# Autodesk Inventor assembly: folivora
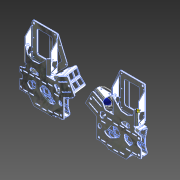
[picture p0: Inventor's stored thumbnail of the model, 180x180]
Saved by Autodesk Inventor 2018 (Build 220112000, 112)
## iProperties
Created: 2018-05-16
Part Number: folivora
Material: 一般
Document SubType Name: Assembly
Designer: NaMACHAN
Mass: 637.628 g
Surface Area: 2506.17 cm^2
Volume: 247.109 cm^3
Density: 2.58035 g/cm^3
Author: NaMACHAN
## Documents named in this file (25)
- C:\Users\NaMACHAN\Dropbox\Project\original\folivora\inventor\folivora.iam
- C:\Users\NaMACHAN\Dropbox\Project\original\folivora\inventor\baseframe.ipt
- C:\Users\NaMACHAN\Dropbox\Project\original\folivora\inventor\keyplate3.ipt
- C:\Users\NaMACHAN\Dropbox\Project\original\folivora\inventor\keyplate4.ipt
- C:\Users\NaMACHAN\Dropbox\Project\original\folivora\inventor\keyL.ipt
- C:\Users\NaMACHAN\Dropbox\Project\original\folivora\inventor\ball.ipt
- C:\Users\NaMACHAN\Dropbox\Project\original\folivora\inventor\trackball-base.ipt
- C:\Users\NaMACHAN\Dropbox\Project\original\folivora\inventor\trackball-shaft.ipt
- C:\Users\NaMACHAN\Dropbox\Project\original\folivora\inventor\bearing.ipt
- C:\Users\NaMACHAN\Dropbox\Project\original\folivora\inventor\bearingcover.ipt
- C:\Users\NaMACHAN\Dropbox\Project\original\folivora\inventor\trackball_l.ipt
- C:\Users\NaMACHAN\Dropbox\Project\original\folivora\inventor\trackball-cover.ipt
- C:\Users\NaMACHAN\Dropbox\Project\original\folivora\inventor\trackball-spacer.ipt
- C:\Users\NaMACHAN\Dropbox\Project\original\folivora\inventor\palmrest.ipt
- C:\Users\NaMACHAN\Dropbox\Project\original\folivora\inventor\palmrest-plate.ipt
- C:\Users\NaMACHAN\Dropbox\Project\original\folivora\inventor\baseframe_left.ipt
- C:\Users\NaMACHAN\Dropbox\Project\original\folivora\inventor\palmrest_left.ipt
- C:\Users\NaMACHAN\Dropbox\Project\original\folivora\inventor\thumbkey_L.ipt
- C:\Users\NaMACHAN\Dropbox\Project\original\folivora\inventor\keyplate2.ipt
- C:\Users\NaMACHAN\Dropbox\Project\original\folivora\inventor\folivora\AIP\FEA\cjjue1qww.fins
- C:\Users\NaMACHAN\Dropbox\Project\original\folivora\inventor\folivora\AIP\FEA\cjjue1qww.fsat
- C:\Users\NaMACHAN\Dropbox\Project\original\folivora\inventor\folivora\AIP\FEA\cjjue1qww.ftes
- C:\Users\NaMACHAN\Dropbox\Project\original\folivora\inventor\folivora\AIP\FEA\cjjue1qww.fwiz
- C:\Users\NaMACHAN\Dropbox\Project\original\folivora\inventor\folivora\AIP\FEA\cjjue1r1c.fmsh
- C:\Users\NaMACHAN\Dropbox\Project\original\folivora\inventor\folivora\AIP\FEA\cjjue1r1d.fres
## Components (61 placed, 18 different names)
1. baseframe:1 — メイト:31, メイト:32, メイト:33, メイト:34, メイト:37, メイト:38, メイト:39, メイト:40, メイト:43, メイト:79, メイト:80, メイト:89, メイト:94, メイト:114, フラッシュ:19, フラッシュ:20, フラッシュ:21, フラッシュ:22, フラッシュ:23, フラッシュ:24, メイト:141, メイト:205, メイト:206, メイト:207
2. keyL:1 — メイト:1, メイト:2, メイト:3, 角度:1, メイト:33
3. keyplate4:1 — メイト:1, メイト:2, メイト:3, メイト:4, メイト:5, 角度:1, メイト:46, メイト:95
4. keyL:2 — メイト:4, メイト:5, メイト:37, メイト:43, フラッシュ:5, フラッシュ:12, フラッシュ:22
5. keyplate3:1 — メイト:6, メイト:7, メイト:8, メイト:9, メイト:10, 角度:2, メイト:44, メイト:45
6. keyL:3 — メイト:7, メイト:10, 角度:2, メイト:32
7. keyL:4 — メイト:6, メイト:8, メイト:9, メイト:40, フラッシュ:3, フラッシュ:4
8. keyplate3:2 — メイト:44
9. keyL:5 — メイト:31
10. keyL:6 — メイト:39, フラッシュ:3
11. keyL:7 — メイト:34
12. keyplate4:2 — メイト:45, メイト:46
13. keyL:8 — メイト:38, フラッシュ:4, フラッシュ:5
14. ball:1 — メイト:105, メイト:115
15. trackball-base:1 — メイト:52, メイト:53, メイト:54, メイト:55, メイト:56, メイト:57, メイト:58, メイト:59, メイト:60, メイト:61, メイト:62, メイト:63, フラッシュ:15, メイト:105, フラッシュ:16, メイト:117, メイト:118, メイト:119, メイト:120, メイト:124, メイト:125
16. trackball-shaft:1 — メイト:49, メイト:52, メイト:53, メイト:54
17. bearing:1 — メイト:49, メイト:55
18. trackball-shaft:2 — メイト:56, メイト:57, メイト:59
19. bearing:2 — メイト:58
20. trackball-shaft:3 — メイト:60, メイト:61, メイト:62
21. bearing:3 — メイト:63
22. bearingcover:1 — フラッシュ:15, フラッシュ:16, メイト:115, メイト:121, メイト:122, メイト:123, メイト:124, メイト:125, メイト:134, メイト:135, メイト:136
23. keyplate3:3 — メイト:140
24. keyL:11 — メイト:80
25. keyL:12 — メイト:79, フラッシュ:13, フラッシュ:21
26. keyL:14 — メイト:89, フラッシュ:12, フラッシュ:13, メイト:93, メイト:200
27. keyL:15 — メイト:94
28. keyplate4:3 — メイト:93, メイト:95, メイト:140, メイト:200
29. trackball_l:1 — メイト:114, メイト:121, メイト:122, メイト:123, フラッシュ:19, フラッシュ:20
30. trackball-shaft:4 — メイト:116, メイト:117, メイト:118, メイト:119
31. bearing:4 — メイト:116, メイト:120
32. trackball-cover:1 — メイト:126, メイト:127, メイト:128, メイト:129, メイト:130, メイト:131, メイト:132, メイト:133
33. trackball-spacer:1 — メイト:126, メイト:130, メイト:136
34. trackball-spacer:2 — メイト:129, メイト:131, メイト:135
35. trackball-spacer:3 — メイト:128, メイト:133
36. trackball-spacer:4 — メイト:127, メイト:132, メイト:134
37. palmrest:1 — メイト:205, メイト:206, メイト:207, メイト:209, メイト:210, メイト:217
38. baseframe_left:1 — フラッシュ:23, フラッシュ:24, メイト:141, メイト:182, メイト:183, メイト:184, メイト:185, メイト:186, メイト:187, メイト:188, メイト:189, メイト:190, メイト:191, メイト:192, メイト:193, フラッシュ:30, フラッシュ:31, メイト:201, フラッシュ:32, フラッシュ:33, メイト:214, メイト:215, メイト:216
39. palmrest_left:1 — メイト:211, メイト:212, メイト:213, メイト:214, メイト:215, メイト:216
40. keyL:16 — メイト:189
41. keyplate4:4 — メイト:196, メイト:197
42. keyL:17 — メイト:183, フラッシュ:31
43. keyplate3:4 — メイト:194, メイト:195
44. keyL:18 — メイト:193
45. keyL:19 — メイト:184
46. keyplate3:5 — メイト:194
47. keyL:20 — メイト:188
48. keyL:21 — メイト:186
49. keyL:22 — メイト:192
50. keyplate4:5 — メイト:195, メイト:196
51. keyL:23 — メイト:185
52. keyplate3:6 — メイト:198
53. keyL:24 — メイト:190
54. keyL:25 — メイト:182, フラッシュ:30
55. keyL:26 — メイト:187, メイト:199
56. keyL:27 — メイト:191
57. keyplate4:6 — メイト:197, メイト:198, メイト:199
58. thumbkey_L:1 — メイト:201, フラッシュ:32, フラッシュ:33, メイト:202, メイト:203, メイト:204
59. keyplate2:1 — メイト:202, メイト:203, メイト:204
60. palmrest-plate:1 — メイト:209, メイト:210, メイト:217
61. palmrest-plate:2 — メイト:211, メイト:212, メイト:213
## Relationships (185: Mate 151, Flush 22, Angle 12)
- メイト:1 [Mate]: keyL:1 ↔ keyplate4:1
- メイト:2 [Mate] (1.5 mm): keyL:1 ↔ keyplate4:1
- メイト:3 [Mate] (15 mm): keyL:1 ↔ keyplate4:1
- メイト:4 [Mate]: keyplate4:1 ↔ keyL:2
- メイト:5 [Mate] (1.5 mm): keyplate4:1 ↔ keyL:2
- メイト:6 [Mate] (1.5 mm): keyplate3:1 ↔ keyL:4
- メイト:7 [Mate]: keyplate3:1 ↔ keyL:3
- メイト:8 [Mate]: keyplate3:1 ↔ keyL:4
- メイト:9 [Mate] (10 mm): keyplate3:1 ↔ keyL:4
- メイト:10 [Mate] (1.5 mm): keyplate3:1 ↔ keyL:3
- 角度:1 [Angle] (0 deg): keyL:1 ↔ keyplate4:1
- 角度:2 [Angle] (0 deg): keyplate3:1 ↔ keyL:3
- [Mate] (1.5 mm): keyplate3:2 ↔ keyL:6
- [Mate]: keyplate3:2 ↔ keyL:5
- [Mate]: keyplate3:2 ↔ keyL:6
- [Mate] (10 mm): keyplate3:2 ↔ keyL:6
- [Mate] (1.5 mm): keyplate3:2 ↔ keyL:5
- [Angle] (0 deg): keyplate3:2 ↔ keyL:5
- [Mate]: keyL:7 ↔ keyplate4:2
- [Mate] (1.5 mm): keyL:7 ↔ keyplate4:2
- [Mate] (15 mm): keyL:7 ↔ keyplate4:2
- [Mate]: keyplate4:2 ↔ keyL:8
- [Mate] (1.5 mm): keyplate4:2 ↔ keyL:8
- [Angle] (0 deg): keyL:7 ↔ keyplate4:2
- メイト:31 [Mate]: baseframe:1 ↔ keyL:5
- メイト:32 [Mate]: baseframe:1 ↔ keyL:3
- メイト:33 [Mate]: baseframe:1 ↔ keyL:1
- メイト:34 [Mate]: baseframe:1 ↔ keyL:7
- メイト:37 [Mate]: baseframe:1 ↔ keyL:2
- メイト:38 [Mate]: baseframe:1 ↔ keyL:8
- メイト:39 [Mate]: baseframe:1 ↔ keyL:6
- メイト:40 [Mate]: baseframe:1 ↔ keyL:4
- メイト:43 [Mate]: baseframe:1 ↔ keyL:2
- フラッシュ:3 [Flush]: keyL:4 ↔ keyL:6
- メイト:44 [Mate]: keyplate3:1 ↔ keyplate3:2
- メイト:45 [Mate]: keyplate3:1 ↔ keyplate4:2
- メイト:46 [Mate]: keyplate4:1 ↔ keyplate4:2
- フラッシュ:4 [Flush] (18 mm): keyL:4 ↔ keyL:8
- フラッシュ:5 [Flush] (3 mm): keyL:2 ↔ keyL:8
- メイト:49 [Mate]: trackball-shaft:1 ↔ bearing:1
- [Mate]: trackball-shaft:2 ↔ bearing:2
- [Mate]: trackball-shaft:3 ↔ bearing:3
- メイト:52 [Mate] (1.5 mm): trackball-base:1 ↔ trackball-shaft:1
- メイト:53 [Mate] (1.5 mm): trackball-base:1 ↔ trackball-shaft:1
- メイト:54 [Mate]: trackball-base:1 ↔ trackball-shaft:1
- メイト:55 [Mate] (0.5 mm): trackball-base:1 ↔ bearing:1
- メイト:56 [Mate] (1.5 mm): trackball-base:1 ↔ trackball-shaft:2
- メイト:57 [Mate] (1.5 mm): trackball-base:1 ↔ trackball-shaft:2
- メイト:58 [Mate] (0.5 mm): trackball-base:1 ↔ bearing:2
- メイト:59 [Mate]: trackball-base:1 ↔ trackball-shaft:2
- メイト:60 [Mate] (1.5 mm): trackball-base:1 ↔ trackball-shaft:3
- メイト:61 [Mate] (1.5 mm): trackball-base:1 ↔ trackball-shaft:3
- メイト:62 [Mate]: trackball-base:1 ↔ trackball-shaft:3
- メイト:63 [Mate] (0.5 mm): trackball-base:1 ↔ bearing:3
- [Mate] (1.5 mm): keyplate3:3 ↔ keyL:12
- [Mate]: keyplate3:3 ↔ keyL:11
- [Mate]: keyplate3:3 ↔ keyL:12
- [Mate] (10 mm): keyplate3:3 ↔ keyL:12
- [Mate] (1.5 mm): keyplate3:3 ↔ keyL:11
- [Angle] (0 deg): keyplate3:3 ↔ keyL:11
- メイト:79 [Mate]: baseframe:1 ↔ keyL:12
- メイト:80 [Mate]: baseframe:1 ↔ keyL:11
- メイト:89 [Mate]: baseframe:1 ↔ keyL:14
- フラッシュ:12 [Flush] (-3 mm): keyL:2 ↔ keyL:14
- フラッシュ:13 [Flush] (3 mm): keyL:12 ↔ keyL:14
- [Mate]: keyL:15 ↔ keyplate4:3
- [Mate] (1.5 mm): keyL:15 ↔ keyplate4:3
- [Mate] (15 mm): keyL:15 ↔ keyplate4:3
- [Angle] (0 deg): keyL:15 ↔ keyplate4:3
- メイト:93 [Mate] (1.5 mm): keyL:14 ↔ keyplate4:3
- メイト:94 [Mate]: baseframe:1 ↔ keyL:15
- メイト:95 [Mate]: keyplate4:1 ↔ keyplate4:3
- フラッシュ:15 [Flush]: trackball-base:1 ↔ bearingcover:1
- メイト:105 [Mate]: ball:1 ↔ trackball-base:1
- メイト:114 [Mate]: baseframe:1 ↔ trackball_l:1
- フラッシュ:16 [Flush]: trackball-base:1 ↔ bearingcover:1
- メイト:115 [Mate] (6.4 mm): ball:1 ↔ bearingcover:1
- メイト:116 [Mate]: trackball-shaft:4 ↔ bearing:4
- メイト:117 [Mate] (1.5 mm): trackball-base:1 ↔ trackball-shaft:4
- メイト:118 [Mate] (1.5 mm): trackball-base:1 ↔ trackball-shaft:4
- メイト:119 [Mate]: trackball-base:1 ↔ trackball-shaft:4
- メイト:120 [Mate] (0.5 mm): trackball-base:1 ↔ bearing:4
- メイト:121 [Mate]: bearingcover:1 ↔ trackball_l:1
- メイト:122 [Mate]: bearingcover:1 ↔ trackball_l:1
- メイト:123 [Mate]: bearingcover:1 ↔ trackball_l:1
- メイト:124 [Mate]: trackball-base:1 ↔ bearingcover:1
- メイト:125 [Mate]: trackball-base:1 ↔ bearingcover:1
- メイト:126 [Mate]: trackball-cover:1 ↔ trackball-spacer:1
- メイト:127 [Mate]: trackball-cover:1 ↔ trackball-spacer:4
- メイト:128 [Mate]: trackball-cover:1 ↔ trackball-spacer:3
- メイト:129 [Mate]: trackball-cover:1 ↔ trackball-spacer:2
- メイト:130 [Mate]: trackball-cover:1 ↔ trackball-spacer:1
- メイト:131 [Mate]: trackball-cover:1 ↔ trackball-spacer:2
- メイト:132 [Mate]: trackball-cover:1 ↔ trackball-spacer:4
- メイト:133 [Mate]: trackball-cover:1 ↔ trackball-spacer:3
- メイト:134 [Mate]: bearingcover:1 ↔ trackball-spacer:4
- メイト:135 [Mate]: bearingcover:1 ↔ trackball-spacer:2
- メイト:136 [Mate]: bearingcover:1 ↔ trackball-spacer:1
- フラッシュ:19 [Flush] (-10 mm): baseframe:1 ↔ trackball_l:1
- フラッシュ:20 [Flush] (-10 mm): baseframe:1 ↔ trackball_l:1
- メイト:140 [Mate]: keyplate3:3 ↔ keyplate4:3
- フラッシュ:21 [Flush] (15 mm): baseframe:1 ↔ keyL:12
- フラッシュ:22 [Flush] (-5 mm): baseframe:1 ↔ keyL:2
- フラッシュ:23 [Flush]: baseframe:1 ↔ baseframe_left:1
- フラッシュ:24 [Flush]: baseframe:1 ↔ baseframe_left:1
- メイト:141 [Mate] (100 mm): baseframe:1 ↔ baseframe_left:1
- [Mate]: keyL:16 ↔ keyplate4:4
- [Mate] (1.5 mm): keyL:16 ↔ keyplate4:4
- [Mate] (15 mm): keyL:16 ↔ keyplate4:4
- [Mate]: keyplate4:4 ↔ keyL:17
- [Mate] (1.5 mm): keyplate4:4 ↔ keyL:17
- [Mate] (1.5 mm): keyplate3:4 ↔ keyL:19
- [Mate]: keyplate3:4 ↔ keyL:18
- [Mate]: keyplate3:4 ↔ keyL:19
- [Mate] (10 mm): keyplate3:4 ↔ keyL:19
- [Mate] (1.5 mm): keyplate3:4 ↔ keyL:18
- [Angle] (0 deg): keyL:16 ↔ keyplate4:4
- [Angle] (0 deg): keyplate3:4 ↔ keyL:18
- [Mate] (1.5 mm): keyplate3:5 ↔ keyL:21
- [Mate]: keyplate3:5 ↔ keyL:20
- [Mate]: keyplate3:5 ↔ keyL:21
- [Mate] (10 mm): keyplate3:5 ↔ keyL:21
- [Mate] (1.5 mm): keyplate3:5 ↔ keyL:20
- [Angle] (0 deg): keyplate3:5 ↔ keyL:20
- [Mate]: keyL:22 ↔ keyplate4:5
- [Mate] (1.5 mm): keyL:22 ↔ keyplate4:5
- [Mate] (15 mm): keyL:22 ↔ keyplate4:5
- [Mate]: keyplate4:5 ↔ keyL:23
- [Mate] (1.5 mm): keyplate4:5 ↔ keyL:23
- [Angle] (0 deg): keyL:22 ↔ keyplate4:5
- [Flush]: keyL:19 ↔ keyL:21
- [Flush] (18 mm): keyL:19 ↔ keyL:23
- [Flush] (3 mm): keyL:17 ↔ keyL:23
- [Mate] (1.5 mm): keyplate3:6 ↔ keyL:25
- [Mate]: keyplate3:6 ↔ keyL:24
- [Mate]: keyplate3:6 ↔ keyL:25
- [Mate] (10 mm): keyplate3:6 ↔ keyL:25
- [Mate] (1.5 mm): keyplate3:6 ↔ keyL:24
- [Angle] (0 deg): keyplate3:6 ↔ keyL:24
- [Flush] (-3 mm): keyL:17 ↔ keyL:26
- [Flush] (3 mm): keyL:25 ↔ keyL:26
- [Mate]: keyL:27 ↔ keyplate4:6
- [Mate] (1.5 mm): keyL:27 ↔ keyplate4:6
- [Mate] (15 mm): keyL:27 ↔ keyplate4:6
- [Angle] (0 deg): keyL:27 ↔ keyplate4:6
- [Mate] (1.5 mm): keyL:26 ↔ keyplate4:6
- メイト:182 [Mate]: baseframe_left:1 ↔ keyL:25
- メイト:183 [Mate]: baseframe_left:1 ↔ keyL:17
- メイト:184 [Mate]: baseframe_left:1 ↔ keyL:19
- メイト:185 [Mate]: baseframe_left:1 ↔ keyL:23
- メイト:186 [Mate]: baseframe_left:1 ↔ keyL:21
- メイト:187 [Mate]: baseframe_left:1 ↔ keyL:26
- メイト:188 [Mate]: baseframe_left:1 ↔ keyL:20
- メイト:189 [Mate]: baseframe_left:1 ↔ keyL:16
- メイト:190 [Mate]: baseframe_left:1 ↔ keyL:24
- メイト:191 [Mate]: baseframe_left:1 ↔ keyL:27
- メイト:192 [Mate]: baseframe_left:1 ↔ keyL:22
- メイト:193 [Mate]: baseframe_left:1 ↔ keyL:18
- メイト:194 [Mate]: keyplate3:4 ↔ keyplate3:5
- メイト:195 [Mate]: keyplate3:4 ↔ keyplate4:5
- メイト:196 [Mate]: keyplate4:4 ↔ keyplate4:5
- メイト:197 [Mate]: keyplate4:4 ↔ keyplate4:6
- メイト:198 [Mate]: keyplate3:6 ↔ keyplate4:6
- メイト:199 [Mate]: keyL:26 ↔ keyplate4:6
- メイト:200 [Mate]: keyL:14 ↔ keyplate4:3
- フラッシュ:30 [Flush] (-10 mm): baseframe_left:1 ↔ keyL:25
- フラッシュ:31 [Flush] (-5 mm): baseframe_left:1 ↔ keyL:17
- メイト:201 [Mate]: baseframe_left:1 ↔ thumbkey_L:1
- フラッシュ:32 [Flush] (12 mm): baseframe_left:1 ↔ thumbkey_L:1
- フラッシュ:33 [Flush]: baseframe_left:1 ↔ thumbkey_L:1
- メイト:202 [Mate]: thumbkey_L:1 ↔ keyplate2:1
- メイト:203 [Mate]: thumbkey_L:1 ↔ keyplate2:1
- メイト:204 [Mate]: thumbkey_L:1 ↔ keyplate2:1
- メイト:205 [Mate]: baseframe:1 ↔ palmrest:1
- メイト:206 [Mate]: baseframe:1 ↔ palmrest:1
- メイト:207 [Mate]: baseframe:1 ↔ palmrest:1
- メイト:209 [Mate]: palmrest:1 ↔ palmrest-plate:1
- メイト:210 [Mate]: palmrest:1 ↔ palmrest-plate:1
- メイト:211 [Mate]: palmrest_left:1 ↔ palmrest-plate:2
- メイト:212 [Mate]: palmrest_left:1 ↔ palmrest-plate:2
- メイト:213 [Mate]: palmrest_left:1 ↔ palmrest-plate:2
- メイト:214 [Mate]: baseframe_left:1 ↔ palmrest_left:1
- メイト:215 [Mate]: baseframe_left:1 ↔ palmrest_left:1
- メイト:216 [Mate]: baseframe_left:1 ↔ palmrest_left:1
- メイト:217 [Mate]: palmrest:1 ↔ palmrest-plate:1
## Named parameters: sa_0 = 7.4e-12, sa_1 = -5000, sa_2 = 4e-13, sa_3 = -1.32e-11, sa_4 = -5000, sa_5 = -4.2e-12, sa_6 = -2.8e-12, sa_7 = -5000, sa_8 = -2.3e-12, sa_9 = -1e-12, sa_10 = -5000, sa_11 = -3.7e-12, sa_12 = 2.78e-11, sa_13 = -5000, sa_14 = 7e-12, sa_15 = 1.85e-11, sa_16 = -5000, sa_17 = 3.9e-12, d377_d369 = 1.5 mm, d378_d370 = 0 mm, d379_d371 = 0 mm, d380_d372 = 10 mm, d381_d373 = 1.5 mm, d382_d375 = 0 deg, d383_d366 = 1.5 mm, d385_d374 = 0 deg, d386_d362 = 0 mm, d387_d363 = 1.5 mm, d388_d364 = 15 mm, d389_d365 = 0 mm, d430_d429 = 0 mm, d431_d429 = 0 mm, d459_d377_d369 = 1.5 mm, d460_d378_d370 = 0 mm, d461_d379_d371 = 0 mm, d462_d380_d372 = 10 mm, d463_d381_d373 = 1.5 mm, d464_d382_d375 = 0 deg, d487_d362 = 0 mm, d488_d363 = 1.5 mm, d489_d364 = 15 mm, d490_d374 = 0 deg, d710_d491 = 1.5 mm, d713_d459_d377_d369 = 1.5 mm, d714_d460_d378_d370 = 0 mm, d715_d461_d379_d371 = 0 mm, d716_d462_d380_d372 = 10 mm, d717_d463_d381_d373 = 1.5 mm, d718_d464_d382_d375 = 0 deg, d719_d481 = -3 mm, d720_d482 = 3 mm, d721_d487_d362 = 0 mm, d722_d488_d363 = 1.5 mm, d723_d489_d364 = 15 mm, d724_d490_d374 = 0 deg, d725_d377_d369 = 1.5 mm, d726_d378_d370 = 0 mm, d727_d379_d371 = 0 mm, d728_d380_d372 = 10 mm, d729_d381_d373 = 1.5 mm, d730_d382_d375 = 0 deg, d731_d383_d366 = 1.5 mm, d732_d385_d374 = 0 deg, d733_d386_d362 = 0 mm, d734_d387_d363 = 1.5 mm, d735_d388_d364 = 15 mm, d736_d389_d365 = 0 mm, d737_d419 = 0 mm, d741_d425 = 18 mm, d742_d426 = 3 mm, d743_d362 = 0 mm, d744_d363 = 1.5 mm, d745_d364 = 15 mm, d746_d365 = 0 mm, d747_d366 = 1.5 mm, d748_d369 = 1.5 mm, d749_d370 = 0 mm, d750_d371 = 0 mm, d751_d372 = 10 mm, d752_d373 = 1.5 mm, d753_d374 = 0 deg, d754_d375 = 0 deg
note: some values were not read from the file. Shown as the stored number, unit unknown: "sa_0", "sa_1", "sa_2", "sa_3", "sa_4", "sa_5", "sa_6", "sa_7", "sa_8", "sa_9", "sa_10", "sa_11", "sa_12", "sa_13", "sa_14", "sa_15", "sa_16", "sa_17".
